# Autodesk Inventor assembly: ENSAMBLE-GARRA
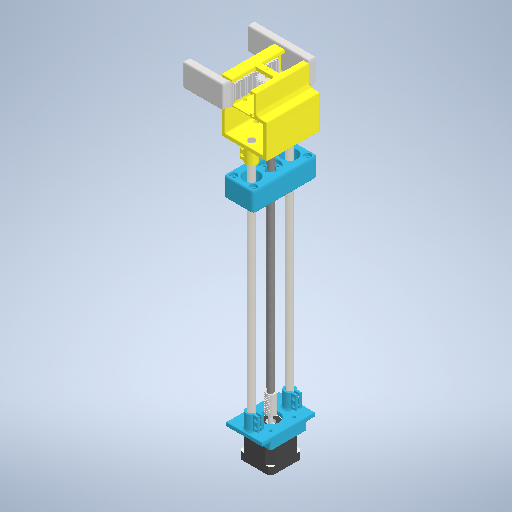
[picture p0: Inventor's stored thumbnail of the model, 512x512]
Saved by Autodesk Inventor 2025.2 (Build 292293000, 293)
## iProperties
Created: 2025-11-05
Part Number: ENSAMBLE-GARRA
Document SubType Name: Assembly
Designer: Jonathan Galarza
Author: Jonathan Galarza
## Documents named in this file (15)
- C:\Users\Dax\Documents\Tesis\MODELADO CAD\GARRA\ENSAMBLE-GARRA.iam
- C:\Users\Dax\Documents\Tesis\MODELADO CAD\GARRA\guia superior.ipt
- C:\Users\Dax\Documents\Tesis\MODELADO CAD\GARRA\Varilla_Redonda.ipt
- C:\Users\Dax\Documents\Tesis\MODELADO CAD\GARRA\baseSup.ipt
- C:\Users\Dax\Documents\Tesis\MODELADO CAD\GARRA\1.Linear Bearing-LM8UU.ipt
- C:\Users\Dax\Documents\Tesis\MODELADO CAD\GARRA\NEMA 17 - MS17HD2.ipt
- C:\Users\Dax\Documents\Tesis\MODELADO CAD\GARRA\tornillo.ipt
- C:\Users\Dax\Documents\Tesis\MODELADO CAD\GARRA\unión.ipt
- C:\Users\Dax\Documents\Tesis\MODELADO CAD\GARRA\baseGuias-motoramarillo.ipt
- C:\Users\Dax\Documents\Tesis\MODELADO CAD\GARRA\chumacera.ipt
- C:\Users\Dax\Documents\Tesis\MODELADO CAD\GARRA\Fitec FS90R Micro Servo NoWires.step.ipt
- C:\Users\Dax\Documents\Tesis\MODELADO CAD\GARRA\piñon-amarillo.ipt
- C:\Users\Dax\Documents\Tesis\MODELADO CAD\GARRA\cremallera 4 - copia.ipt
- C:\Users\Dax\Documents\Tesis\MODELADO CAD\GARRA\cremallera 4.ipt
- C:\Users\Dax\Documents\Tesis\MODELADO CAD\GARRA\NEMA 17 - MS17HD2\NEMA 17 - MS17HD2\NEMA 17 - MS17HD2.ipt
## Components (16 placed, 13 different names)
1. guia superior:1 — Coincidencia:11, Coincidencia:12
2. Varilla_Redonda:1 — Coincidencia:7, Nivelación:2, Coincidencia:12, Nivelación:5, Coincidencia:13
3. Varilla_Redonda:2 — Coincidencia:5, Coincidencia:6, Nivelación:3, Coincidencia:11, Nivelación:4
4. baseSup:1 — Coincidencia:3, Coincidencia:6, Coincidencia:7, Nivelación:2, Nivelación:3, Coincidencia:8, Coincidencia:9, Coincidencia:10
5. 1.Linear Bearing-LM8UU:1
6. 1.Linear Bearing-LM8UU:2
7. NEMA 17 - MS17HD2:1 — Coincidencia:3, Coincidencia:4, Nivelación:1
8. tornillo:1 — Coincidencia:14, Coincidencia:17, Coincidencia:18
9. unión:1 — Coincidencia:4, Nivelación:1, Coincidencia:16, Coincidencia:18
10. baseGuias-motoramarillo:1 — Coincidencia:5, Nivelación:4, Nivelación:5, Coincidencia:13, Coincidencia:15, Coincidencia:19, Coincidencia:20, Coincidencia:21, Coincidencia:22, Coincidencia:23, Coincidencia:24, Coincidencia:25
11. chumacera:1 — Coincidencia:14, Coincidencia:15
12. Fitec FS90R Micro Servo NoWires.step:1 — Insertar:13, Coincidencia:23, Coincidencia:24, Coincidencia:25
13. piñon-amarillo:1 — Insertar:13, Rotación/Traslación:1, Rotación/Traslación:2
14. cremallera 4 - copia:1 — Rotación/Traslación:2, Coincidencia:19, Coincidencia:20
15. cremallera 4:1 — Rotación/Traslación:1, Coincidencia:21, Coincidencia:22
16. NEMA 17 - MS17HD2:2 — Coincidencia:8, Coincidencia:9, Coincidencia:10, Coincidencia:16, Coincidencia:17
## Relationships (31: Mate 23, Flush 5, RelateRotateTranslate 2, Insert 1)
- Coincidencia:3 [Mate]: baseSup:1 ↔ NEMA 17 - MS17HD2:1
- Coincidencia:4 [Mate]: NEMA 17 - MS17HD2:1 ↔ unión:1
- Nivelación:1 [Flush]: NEMA 17 - MS17HD2:1 ↔ unión:1
- Insertar:13: Fitec FS90R Micro Servo NoWires.step:1 ↔ piñon-amarillo:1
- Rotación/Traslación:1 [RelateRotateTranslate] (62.8 mm): piñon-amarillo:1 ↔ cremallera 4:1
- Rotación/Traslación:2 [RelateRotateTranslate] (62.8 mm): piñon-amarillo:1 ↔ cremallera 4 - copia:1
- Coincidencia:5 [Mate]: Varilla_Redonda:2 ↔ baseGuias-motoramarillo:1
- Coincidencia:6 [Mate]: Varilla_Redonda:2 ↔ baseSup:1
- Coincidencia:7 [Mate]: Varilla_Redonda:1 ↔ baseSup:1
- Nivelación:2 [Flush]: Varilla_Redonda:1 ↔ baseSup:1
- Nivelación:3 [Flush]: Varilla_Redonda:2 ↔ baseSup:1
- Coincidencia:8 [Mate]: baseSup:1 ↔ NEMA 17 - MS17HD2:2
- Coincidencia:9 [Mate]: baseSup:1 ↔ NEMA 17 - MS17HD2:2
- Coincidencia:10 [Mate]: baseSup:1 ↔ NEMA 17 - MS17HD2:2
- Coincidencia:11 [Mate]: guia superior:1 ↔ Varilla_Redonda:2
- Coincidencia:12 [Mate]: guia superior:1 ↔ Varilla_Redonda:1
- Nivelación:4 [Flush]: Varilla_Redonda:2 ↔ baseGuias-motoramarillo:1
- Nivelación:5 [Flush]: Varilla_Redonda:1 ↔ baseGuias-motoramarillo:1
- Coincidencia:13 [Mate]: Varilla_Redonda:1 ↔ baseGuias-motoramarillo:1
- Coincidencia:14 [Mate]: tornillo:1 ↔ chumacera:1
- Coincidencia:15 [Mate]: baseGuias-motoramarillo:1 ↔ chumacera:1
- Coincidencia:16 [Mate]: unión:1 ↔ NEMA 17 - MS17HD2:2
- Coincidencia:17 [Mate]: tornillo:1 ↔ NEMA 17 - MS17HD2:2
- Coincidencia:18 [Mate]: tornillo:1 ↔ unión:1
- Coincidencia:19 [Mate]: baseGuias-motoramarillo:1 ↔ cremallera 4 - copia:1
- Coincidencia:20 [Mate]: baseGuias-motoramarillo:1 ↔ cremallera 4 - copia:1
- Coincidencia:21 [Mate]: baseGuias-motoramarillo:1 ↔ cremallera 4:1
- Coincidencia:22 [Mate]: baseGuias-motoramarillo:1 ↔ cremallera 4:1
- Coincidencia:23 [Mate]: baseGuias-motoramarillo:1 ↔ Fitec FS90R Micro Servo NoWires.step:1
- Coincidencia:24 [Mate]: baseGuias-motoramarillo:1 ↔ Fitec FS90R Micro Servo NoWires.step:1
- Coincidencia:25 [Mate]: baseGuias-motoramarillo:1 ↔ Fitec FS90R Micro Servo NoWires.step:1
